# Autodesk Inventor assembly: Сборка1
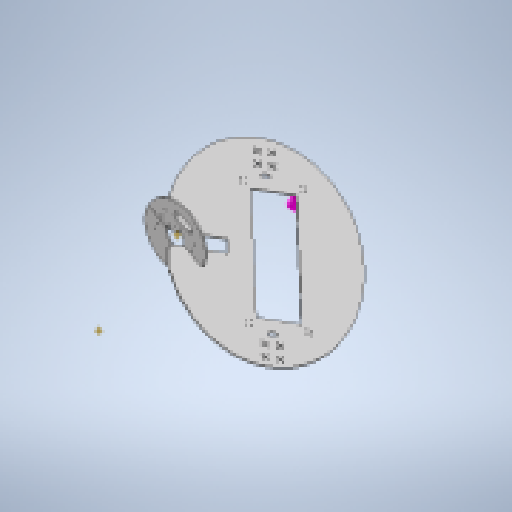
[picture p0: Inventor's stored thumbnail of the model, 512x512]
Saved by Autodesk Inventor 2023.1 (Build 271208000, 208)
## iProperties
Created: 2025-02-03
Part Number: Сборка1
Document SubType Name: Assembly
Designer: baranovaem
Author: baranovaem
## Documents named in this file (5)
- C:\Users\DELL\reposGitHub\Cheburashka\Cheburashka_construction\face\лицо\Сборка1.iam
- C:\Users\DELL\reposGitHub\Cheburashka\Cheburashka_construction\face\лицо\магнит_стойка.ipt
- C:\Users\DELL\reposGitHub\Cheburashka\Cheburashka_construction\face\лицо\монитор.ipt
- C:\Users\DELL\reposGitHub\Cheburashka\Cheburashka_construction\face\лицо\основа_лица.ipt
- C:\Users\DELL\reposGitHub\Cheburashka\Cheburashka_construction\face\лицо\лицо1.ipt
## Components (5 placed, 4 different names)
1. магнит_стойка:2 — Совмещение:91, Совмещение:92, Совмещение:93, Совмещение:100, Совмещение:101
2. магнит_стойка:4 — Совмещение:89, Совмещение:90, Совмещение:94, Совмещение:102
3. монитор:1 — Совмещение:100, Совмещение:101, Совмещение:102
4. основа_лица:1 — Совмещение:89, Совмещение:90, Совмещение:91, Совмещение:92, Совмещение:93, Совмещение:94, Совмещение:103, Совмещение:104, Совмещение:105
5. лицо1:1 — Совмещение:103, Совмещение:104, Совмещение:105
## Relationships (12: Mate 12)
- Совмещение:89 [Mate]: магнит_стойка:4 ↔ основа_лица:1
- Совмещение:90 [Mate]: магнит_стойка:4 ↔ основа_лица:1
- Совмещение:91 [Mate]: магнит_стойка:2 ↔ основа_лица:1
- Совмещение:92 [Mate]: магнит_стойка:2 ↔ основа_лица:1
- Совмещение:93 [Mate]: магнит_стойка:2 ↔ основа_лица:1
- Совмещение:94 [Mate]: магнит_стойка:4 ↔ основа_лица:1
- Совмещение:100 [Mate]: магнит_стойка:2 ↔ монитор:1
- Совмещение:101 [Mate]: магнит_стойка:2 ↔ монитор:1
- Совмещение:102 [Mate]: магнит_стойка:4 ↔ монитор:1
- Совмещение:103 [Mate]: основа_лица:1 ↔ лицо1:1
- Совмещение:104 [Mate]: основа_лица:1 ↔ лицо1:1
- Совмещение:105 [Mate]: основа_лица:1 ↔ лицо1:1
